# Autodesk Inventor assembly: gas shock
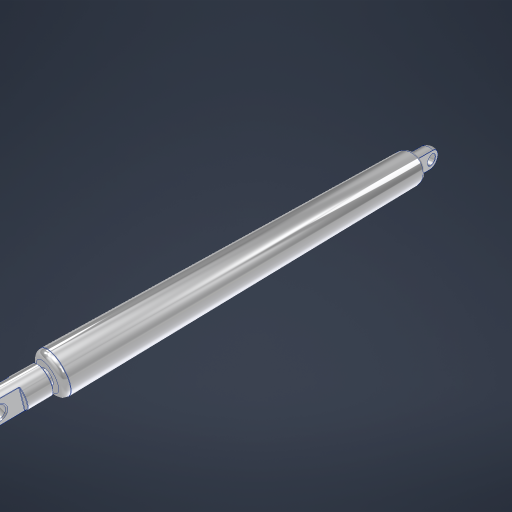
[picture p0: Inventor's stored thumbnail of the model, 512x512]
Saved by Autodesk Inventor 2023.4 (Build 274418000, 418)
## iProperties
Created: 2025-03-21
Part Number: gas shock
Document SubType Name: Assembly
Designer: brand
Mass: 81.9301 g
Surface Area: 144.892 cm^2
Volume: 33.1093 cm^3
Author: brand
## Documents named in this file (3)
- C:\Users\brand\OneDrive\Documents\GitHub\robotics 23\2025-ReefScape---CAD\COMMON PARTS\Z - STEPS\4253N131_Gas Spring with Eyelet Fittings\gas shock.iam
- C:\Users\brand\OneDrive\Documents\GitHub\robotics 23\2025-ReefScape---CAD\COMMON PARTS\Z - STEPS\4253N131_Gas Spring with Eyelet Fittings\cyl 4253N131_Gas Spring with Eyelet Fittings.ipt
- C:\Users\brand\OneDrive\Documents\GitHub\robotics 23\2025-ReefScape---CAD\COMMON PARTS\Z - STEPS\4253N131_Gas Spring with Eyelet Fittings\rod 4253N131_Gas Spring with Eyelet Fittings.ipt
## Components (2 placed, 2 different names)
1. cyl 4253N131_Gas Spring with Eyelet Fittings:1 — Insert:1, Angle:1
2. rod 4253N131_Gas Spring with Eyelet Fittings:1 — Insert:1, Angle:1
## Relationships (2: Insert 1, Angle 1)
- Insert:1 (-2.794 mm): cyl 4253N131_Gas Spring with Eyelet Fittings:1 ↔ rod 4253N131_Gas Spring with Eyelet Fittings:1
- Angle:1 (0 deg): cyl 4253N131_Gas Spring with Eyelet Fittings:1 ↔ rod 4253N131_Gas Spring with Eyelet Fittings:1
